# Autodesk Inventor assembly: capit
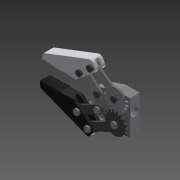
[picture p0: Inventor's stored thumbnail of the model, 180x180]
Saved by Autodesk Inventor 2019 (Build 230136000, 136)
## iProperties
Created: 2016-12-05
Part Number: capit
Document SubType Name: Assembly
Designer: MuhammadArdian
Author: MuhammadArdian
## Documents named in this file (7)
- D:\Kuliah\Sem 1\Workshop Gambar Teknik\Inventor\Latihan Pertemuan 12 - Robotic Arm\capit.iam
- D:\Kuliah\Sem 1\Workshop Gambar Teknik\Inventor\Latihan Pertemuan 12 - Robotic Arm\gerigi.ipt
- D:\Kuliah\Sem 1\Workshop Gambar Teknik\Inventor\Latihan Pertemuan 12 - Robotic Arm\penompang capit.ipt
- D:\Kuliah\Sem 1\Workshop Gambar Teknik\Inventor\Latihan Pertemuan 12 - Robotic Arm\Sendi Capit.ipt
- D:\Kuliah\Sem 1\Workshop Gambar Teknik\Inventor\Latihan Pertemuan 12 - Robotic Arm\Telapak.ipt
- D:\Kuliah\Sem 1\Workshop Gambar Teknik\Inventor\Latihan Pertemuan 12 - Robotic Arm\capit.ipt
- D:\Kuliah\Sem 1\Workshop Gambar Teknik\Inventor\Latihan Pertemuan 12 - Robotic Arm\Mur Sendi Capit.ipt
## Components (23 placed, 6 different names)
1. gerigi:1 — Mate:9, Mate:11, Mate:19, Mate:28, Mate:48, Rotation:1
2. penompang capit:1 — Mate:14, Mate:16, Mate:17, Mate:47
3. Sendi Capit:1 — Mate:1, Mate:5, Mate:10, Mate:37, Mate:38
4. Telapak:1 — Mate:1, Mate:2, Mate:3, Mate:4, Mate:5, Mate:6, Mate:7, Mate:8, Mate:11, Mate:12, Mate:15, Mate:16
5. Sendi Capit:2 — Mate:3, Mate:7, Mate:9, Mate:35, Mate:36
6. Sendi Capit:3 — Mate:2, Mate:6, Mate:13, Mate:39, Mate:40
7. Sendi Capit:4 — Mate:4, Mate:8, Mate:14, Mate:33, Mate:34
8. gerigi:2 — Mate:10, Mate:12, Mate:21, Mate:49, Rotation:1
9. penompang capit:2 — Mate:13, Mate:15, Mate:24, Mate:25, Mate:52
10. Sendi Capit:5 — Mate:17, Mate:27, Mate:31, Mate:32
11. Sendi Capit:6 — Mate:19, Mate:26, Mate:29, Mate:30
12. Sendi Capit:8 — Mate:21, Mate:23, Mate:41, Mate:42
13. Sendi Capit:9 — Mate:22, Mate:24, Mate:43, Mate:44
14. capit:1 — Mate:22, Mate:23, Mate:25, Mate:50, Mate:51
15. capit:2 — Mate:26, Mate:27, Mate:28, Mate:45, Mate:46
16. Mur Sendi Capit:1 — Mate:31, Mate:32, Mate:45
17. Mur Sendi Capit:2 — Mate:29, Mate:30, Mate:46
18. Mur Sendi Capit:3 — Mate:33, Mate:34, Mate:47
19. Mur Sendi Capit:4 — Mate:35, Mate:36, Mate:48
20. Mur Sendi Capit:5 — Mate:37, Mate:38, Mate:49
21. Mur Sendi Capit:6 — Mate:39, Mate:40, Mate:52
22. Mur Sendi Capit:7 — Mate:41, Mate:42, Mate:51
23. Mur Sendi Capit:8 — Mate:43, Mate:44, Mate:50
## Relationships (51: Mate 50, RelateRotation 1)
- Mate:1: Sendi Capit:1 ↔ Telapak:1
- Mate:2: Telapak:1 ↔ Sendi Capit:3
- Mate:3: Telapak:1 ↔ Sendi Capit:2
- Mate:4: Telapak:1 ↔ Sendi Capit:4
- Mate:5: Sendi Capit:1 ↔ Telapak:1
- Mate:6: Telapak:1 ↔ Sendi Capit:3
- Mate:7: Telapak:1 ↔ Sendi Capit:2
- Mate:8: Telapak:1 ↔ Sendi Capit:4
- Mate:9: gerigi:1 ↔ Sendi Capit:2
- Mate:10: Sendi Capit:1 ↔ gerigi:2
- Mate:11: gerigi:1 ↔ Telapak:1
- Mate:12: Telapak:1 ↔ gerigi:2
- Mate:13: Sendi Capit:3 ↔ penompang capit:2
- Mate:14: penompang capit:1 ↔ Sendi Capit:4
- Mate:15: Telapak:1 ↔ penompang capit:2
- Mate:16: penompang capit:1 ↔ Telapak:1
- Mate:17: penompang capit:1 ↔ Sendi Capit:5
- Mate:19: gerigi:1 ↔ Sendi Capit:6
- Mate:21: gerigi:2 ↔ Sendi Capit:8
- Mate:22: Sendi Capit:9 ↔ capit:1
- Mate:23: Sendi Capit:8 ↔ capit:1
- Mate:24: penompang capit:2 ↔ Sendi Capit:9
- Mate:25: penompang capit:2 ↔ capit:1
- Mate:26: Sendi Capit:6 ↔ capit:2
- Mate:27: Sendi Capit:5 ↔ capit:2
- Mate:28: gerigi:1 ↔ capit:2
- Mate:29: Sendi Capit:6 ↔ Mur Sendi Capit:2
- Mate:30: Sendi Capit:6 ↔ Mur Sendi Capit:2
- Mate:31: Sendi Capit:5 ↔ Mur Sendi Capit:1
- Mate:32: Sendi Capit:5 ↔ Mur Sendi Capit:1
- Mate:33: Sendi Capit:4 ↔ Mur Sendi Capit:3
- Mate:34: Sendi Capit:4 ↔ Mur Sendi Capit:3
- Mate:35: Sendi Capit:2 ↔ Mur Sendi Capit:4
- Mate:36: Sendi Capit:2 ↔ Mur Sendi Capit:4
- Mate:37: Sendi Capit:1 ↔ Mur Sendi Capit:5
- Mate:38: Sendi Capit:1 ↔ Mur Sendi Capit:5
- Mate:39: Sendi Capit:3 ↔ Mur Sendi Capit:6
- Mate:40: Sendi Capit:3 ↔ Mur Sendi Capit:6
- Mate:41: Sendi Capit:8 ↔ Mur Sendi Capit:7
- Mate:42: Sendi Capit:8 ↔ Mur Sendi Capit:7
- Mate:43: Sendi Capit:9 ↔ Mur Sendi Capit:8
- Mate:44: Sendi Capit:9 ↔ Mur Sendi Capit:8
- Mate:45: capit:2 ↔ Mur Sendi Capit:1
- Mate:46: capit:2 ↔ Mur Sendi Capit:2
- Mate:47: penompang capit:1 ↔ Mur Sendi Capit:3
- Mate:48: gerigi:1 ↔ Mur Sendi Capit:4
- Mate:49: gerigi:2 ↔ Mur Sendi Capit:5
- Mate:50: capit:1 ↔ Mur Sendi Capit:8
- Mate:51: capit:1 ↔ Mur Sendi Capit:7
- Mate:52: penompang capit:2 ↔ Mur Sendi Capit:6
- Rotation:1 [RelateRotation] (1 ul): gerigi:1 ↔ gerigi:2
